# Autodesk Inventor assembly: Ensamblaje gibox v1.3
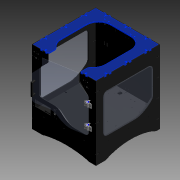
[picture p0: Inventor's stored thumbnail of the model, 180x180]
Saved by Autodesk Inventor 2012 SP1 (Build 160190100, 190)
## iProperties
Created: 2015-03-29
Part Number: Ensamblaje gibox v1.3
Document SubType Name: Assembly
Designer: sheina
Author: sheina
## Documents named in this file (12)
- C:\Users\Laser router cnc\Desktop\compartir con principal\impresora juan marc albert\Ultima modificacio Impresora\modificacio chasis 1-9-14\Ensamblaje gibox v1.3.iam
- C:\Users\Laser router cnc\Desktop\compartir con principal\impresora juan marc albert\Ultima modificacio Impresora\modificacio chasis 1-9-14\base.ipt
- C:\Users\Laser router cnc\Desktop\compartir con principal\impresora juan marc albert\Ultima modificacio Impresora\modificacio chasis 1-9-14\esquena.ipt
- C:\Users\Laser router cnc\Desktop\compartir con principal\impresora juan marc albert\Ultima modificacio Impresora\modificacio chasis 1-9-14\lateral esquerra.ipt
- C:\Users\Laser router cnc\Desktop\compartir con principal\impresora juan marc albert\Ultima modificacio Impresora\modificacio chasis 1-9-14\lateral dret.ipt
- C:\Users\Laser router cnc\Desktop\compartir con principal\impresora juan marc albert\Ultima modificacio Impresora\modificacio chasis 1-9-14\pieza frontal nueva.ipt
- C:\Users\Laser router cnc\Desktop\compartir con principal\impresora juan marc albert\Ultima modificacio Impresora\modificacio chasis 1-9-14\sostre.ipt
- C:\Users\Laser router cnc\Desktop\compartir con principal\impresora juan marc albert\Ultima modificacio Impresora\modificacio chasis 1-9-14\metacrilat proteccio esquerra.ipt
- C:\Users\Laser router cnc\Desktop\compartir con principal\impresora juan marc albert\Ultima modificacio Impresora\modificacio chasis 1-9-14\metacrilat proteccio dret.ipt
- C:\Users\Laser router cnc\Desktop\compartir con principal\impresora juan marc albert\Ultima modificacio Impresora\modificacio chasis 1-9-14\porta frontal.ipt
- C:\Users\Laser router cnc\Desktop\compartir con principal\impresora juan marc albert\Ultima modificacio Impresora\modificacio chasis 1-9-14\frontissa.iam
- C:\Users\Laser router cnc\Desktop\compartir con principal\impresora juan marc albert\Ultima modificacio Impresora\modificacio chasis 1-9-14\maneta porta.ipt
## Components (12 placed, 11 different names)
1. base:1 — Nivelación:1, Nivelación:2, Coincidencia:1, Coincidencia:2, Coincidencia:3, Nivelación:3
2. esquena:1 — Nivelación:1, Nivelación:2, Coincidencia:1, Coincidencia:4, Nivelación:7
3. lateral dret:1 — Coincidencia:6, Nivelación:6, Nivelación:7, Coincidencia:9, Nivelación:14
4. pieza frontal nueva:1 — Coincidencia:2, Coincidencia:3, Nivelación:3, Coincidencia:5, Nivelación:4, Nivelación:10, Nivelación:11, Nivelación:13, Insertar:5, Insertar:6, Insertar:7, Insertar:8
5. sostre:1 — Coincidencia:4, Coincidencia:5, Nivelación:4, Coincidencia:6, Nivelación:6, Coincidencia:7, Nivelación:9, Nivelación:12
6. lateral esquerra:2 — Coincidencia:7, Nivelación:9, Nivelación:10, Coincidencia:8
7. metacrilat proteccio esquerra:1 — Nivelación:11, Nivelación:12, Coincidencia:8
8. metacrilat proteccio dret:1 — Coincidencia:9, Nivelación:13, Nivelación:14
9. porta frontal:1 — Insertar:1, Insertar:2, Insertar:3, Insertar:4, Insertar:9, Insertar:10
10. frontissa:1 [sub-assembly] — Insertar:1, Insertar:2, Insertar:5, Insertar:6
11. frontissa:2 [sub-assembly] — Insertar:3, Insertar:4, Insertar:7, Insertar:8
12. maneta porta:1 — Insertar:9, Insertar:10
## Relationships (31: Flush 12, Insert 10, Mate 9)
- Nivelación:1 [Flush]: base:1 ↔ esquena:1
- Nivelación:2 [Flush]: base:1 ↔ esquena:1
- Coincidencia:1 [Mate]: base:1 ↔ esquena:1
- Coincidencia:2 [Mate]: base:1 ↔ pieza frontal nueva:1
- Coincidencia:3 [Mate]: base:1 ↔ pieza frontal nueva:1
- Nivelación:3 [Flush]: base:1 ↔ pieza frontal nueva:1
- Coincidencia:4 [Mate]: esquena:1 ↔ sostre:1
- Coincidencia:5 [Mate]: pieza frontal nueva:1 ↔ sostre:1
- Nivelación:4 [Flush]: pieza frontal nueva:1 ↔ sostre:1
- Coincidencia:6 [Mate]: lateral dret:1 ↔ sostre:1
- Nivelación:6 [Flush]: lateral dret:1 ↔ sostre:1
- Nivelación:7 [Flush]: esquena:1 ↔ lateral dret:1
- Coincidencia:7 [Mate]: sostre:1 ↔ lateral esquerra:2
- Nivelación:9 [Flush]: sostre:1 ↔ lateral esquerra:2
- Nivelación:10 [Flush]: pieza frontal nueva:1 ↔ lateral esquerra:2
- Nivelación:11 [Flush] (44 mm): pieza frontal nueva:1 ↔ metacrilat proteccio esquerra:1
- Nivelación:12 [Flush] (83 mm): sostre:1 ↔ metacrilat proteccio esquerra:1
- Coincidencia:8 [Mate]: lateral esquerra:2 ↔ metacrilat proteccio esquerra:1
- Coincidencia:9 [Mate]: lateral dret:1 ↔ metacrilat proteccio dret:1
- Nivelación:13 [Flush] (44 mm): pieza frontal nueva:1 ↔ metacrilat proteccio dret:1
- Nivelación:14 [Flush] (-83 mm): lateral dret:1 ↔ metacrilat proteccio dret:1
- Insertar:1: porta frontal:1 ↔ frontissa:1
- Insertar:2: porta frontal:1 ↔ frontissa:1
- Insertar:3: porta frontal:1 ↔ frontissa:2
- Insertar:4: porta frontal:1 ↔ frontissa:2
- Insertar:5: pieza frontal nueva:1 ↔ frontissa:1
- Insertar:6: pieza frontal nueva:1 ↔ frontissa:1
- Insertar:7: pieza frontal nueva:1 ↔ frontissa:2
- Insertar:8: pieza frontal nueva:1 ↔ frontissa:2
- Insertar:9: porta frontal:1 ↔ maneta porta:1
- Insertar:10: porta frontal:1 ↔ maneta porta:1
